(part 1 of 3)
# Autodesk Inventor assembly: Почти готово_CPY
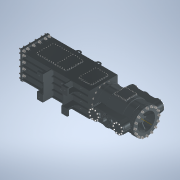
[picture p0: Inventor's stored thumbnail of the model, 180x180]
Saved by Autodesk Inventor 2021 (Build 250183000, 183)
## iProperties
Created: 2020-12-08
Part Number: Почти готово_CPY
Document SubType Name: Assembly
Designer: Тимоха
Author: Тимоха
## Documents named in this file (74)
- C:\Users\Тимоха\Desktop\КР Компрессор\compressor\Почти готово_CPY.iam
- C:\Users\Тимоха\Desktop\КР Компрессор\compressor\Фонарь_CPY.ipt
- C:\Users\Тимоха\Desktop\КР Компрессор\compressor\Башмак_CPY.ipt
- C:\Users\Тимоха\Desktop\КР Компрессор\compressor\Втулка палец шатун_CPY.ipt
- C:\Users\Тимоха\Desktop\КР Компрессор\compressor\Втулка под палец_CPY.ipt
- C:\Users\Тимоха\Desktop\КР Компрессор\compressor\Гайка шток_CPY.ipt
- C:\Users\Тимоха\Desktop\КР Компрессор\compressor\Крейцкопф_CPY.ipt
- C:\Users\Тимоха\Desktop\КР Компрессор\compressor\Палец_CPY.ipt
- C:\Users\Тимоха\Desktop\КР Компрессор\compressor\Стопорное кольцо_CPY.ipt
- C:\Users\Тимоха\Desktop\КР Компрессор\compressor\Верхняя часть поршня_CPY.ipt
- C:\Users\Тимоха\Desktop\КР Компрессор\compressor\Втулка_CPY.ipt
- C:\Users\Тимоха\Desktop\КР Компрессор\compressor\Гайка шток-поршень_CPY.ipt
- C:\Users\Тимоха\Desktop\КР Компрессор\compressor\Кольцо поршень-шток верх_CPY.ipt
- C:\Users\Тимоха\Desktop\КР Компрессор\compressor\Кольцо поршень-шток низ_CPY.ipt
- C:\Users\Тимоха\Desktop\КР Компрессор\compressor\Кольцо поршня_CPY.ipt
- C:\Users\Тимоха\Desktop\КР Компрессор\compressor\Кольцо сальника_CPY.ipt
- C:\Users\Тимоха\Desktop\КР Компрессор\compressor\Корпус дросселя_CPY.ipt
- C:\Users\Тимоха\Desktop\КР Компрессор\compressor\Корпус сальника_CPY.ipt
- C:\Users\Тимоха\Desktop\КР Компрессор\compressor\Крышка стакана_CPY.ipt
- C:\Users\Тимоха\Desktop\КР Компрессор\compressor\Крышка цилиндра 1_CPY.ipt
- C:\Users\Тимоха\Desktop\КР Компрессор\compressor\Крышка цилиндра 2_CPY.ipt
- C:\Users\Тимоха\Desktop\КР Компрессор\compressor\Нижняя часть поршня_CPY.ipt
- C:\Users\Тимоха\Desktop\КР Компрессор\compressor\Опорное кольцо_CPY.ipt
- C:\Users\Тимоха\Desktop\КР Компрессор\compressor\Пружина дросселя_CPY.ipt
- C:\Users\Тимоха\Desktop\КР Компрессор\compressor\Пружина сальника_CPY.ipt
- C:\Users\Тимоха\Desktop\КР Компрессор\compressor\Цилиндр2_CPY.ipt
- C:\Users\Тимоха\Desktop\КР Компрессор\compressor\Клапан1_CPY.iam
- C:\Users\Тимоха\Desktop\КР Компрессор\compressor\Прокладка клапана_CPY.ipt
- C:\Users\Тимоха\Desktop\КР Компрессор\compressor\Стакан1_CPY.ipt
- C:\Users\Тимоха\Desktop\КР Компрессор\compressor\Дроссельное кольцо_CPY.ipt
- C:\Users\Тимоха\Desktop\КР Компрессор\compressor\Уплотнительное кольцо_CPY.ipt
- C:\Users\Тимоха\Desktop\КР Компрессор\compressor\Уплотнение фонарь_CPY.ipt
- C:\Users\Тимоха\Desktop\КР Компрессор\compressor\Крышка сальников_CPY.ipt
- C:\Users\Тимоха\Desktop\КР Компрессор\compressor\Корпус маслосъемника_CPY.ipt
- C:\Users\Тимоха\Desktop\КР Компрессор\compressor\Корпус сальника перегородка 1_CPY.ipt
- C:\Users\Тимоха\Desktop\КР Компрессор\compressor\Крышка перегородки11_CPY.ipt
- C:\Users\Тимоха\Desktop\КР Компрессор\compressor\Крышка перегородки12_CPY.ipt
- C:\Users\Тимоха\Desktop\КР Компрессор\compressor\Крышка перегородки21_CPY.ipt
- C:\Users\Тимоха\Desktop\КР Компрессор\compressor\Крышка перегородки22_CPY.ipt
- C:\Users\Тимоха\Desktop\КР Компрессор\compressor\Маслосъемная пружина_CPY.ipt
- C:\Users\Тимоха\Desktop\КР Компрессор\compressor\Маслосъемное кольцо_CPY.ipt
- C:\Users\Тимоха\Desktop\КР Компрессор\compressor\Придав перегородки1_CPY.ipt
- C:\Users\Тимоха\Desktop\КР Компрессор\compressor\Фланецгайка_CPY.ipt
- C:\Users\Тимоха\Desktop\КР Компрессор\compressor\Шток_CPY.ipt
- C:\Users\Тимоха\Desktop\КР Компрессор\compressor\Прокладка крейцкопф_CPY.ipt
- C:\Users\Тимоха\Documents\Inventor\Content Center Files\R2021\ru-RU\Stud GOST 22038-76\Шпилька M24-6g×70 ГОСТ 22038-76.ipt
- C:\Users\Тимоха\Documents\Inventor\Content Center Files\R2021\ru-RU\Nut GOST 15524-70\Гайка M24-6H ГОСТ 15524-70.ipt
- C:\Users\Тимоха\Documents\Inventor\Content Center Files\R2021\ru-RU\GOST 11371-78  A\Шайба 24 ГОСТ 11371-78.ipt
- C:\Users\Тимоха\Documents\Inventor\Content Center Files\R2021\ru-RU\GOST 15521-70\Гайка M20-6H ГОСТ 15521-70.ipt
- C:\Users\Тимоха\Documents\Inventor\Content Center Files\R2021\ru-RU\Stud GOST 22034-76\Шпилька M20-6g×50 ГОСТ 22034-76.ipt
- C:\Users\Тимоха\Documents\Inventor\Content Center Files\R2021\ru-RU\GOST 10450-78\Шайба 19 ГОСТ 10450-78.ipt
- C:\Users\Тимоха\Documents\Inventor\Content Center Files\R2021\ru-RU\Stud GOST 22038-76\Шпилька M20-6g×85 ГОСТ 22038-76.ipt
- C:\Users\Тимоха\Documents\Inventor\Content Center Files\R2021\ru-RU\GOST 10450-78\Шайба 21 ГОСТ 10450-78.ipt
- C:\Users\Тимоха\Documents\Inventor\Content Center Files\R2021\ru-RU\Nut GOST 15524-70\Гайка M20-6H ГОСТ 15524-70.ipt
- C:\Users\Тимоха\Documents\Inventor\Content Center Files\R2021\ru-RU\GOST 11738-84\Винт M10-6gx35 ГОСТ 11738-84.ipt
- C:\Users\Тимоха\Documents\Inventor\Content Center Files\R2021\ru-RU\GOST 11371-78  A\Шайба 12 ГОСТ 11371-78.ipt
- C:\Users\Тимоха\Documents\Inventor\Content Center Files\R2021\ru-RU\GOST 11738-84\Винт M10-6gx30 ГОСТ 11738-84.ipt
- C:\Users\Тимоха\Documents\Inventor\Content Center Files\R2021\ru-RU\GOST 11738-84\Винт M10-6gx25 ГОСТ 11738-84.ipt
- C:\Users\Тимоха\Documents\Inventor\Content Center Files\R2021\ru-RU\Stud GOST 22038-76\Шпилька M24-6g×80 ГОСТ 22038-76.ipt
- C:\Users\Тимоха\Documents\Inventor\Content Center Files\R2021\ru-RU\GOST 11371-78  A\Шайба 27 ГОСТ 11371-78.ipt
- C:\Users\Тимоха\Desktop\КР Компрессор\compressor\Крышка стакана_MIR_CPY.ipt
- C:\Users\Тимоха\Desktop\КР Компрессор\compressor\Деталь5_CPY.ipt
- C:\Users\Тимоха\Desktop\КР Компрессор\compressor\Деталь6_CPY.ipt
- C:\Users\Тимоха\Documents\Inventor\Content Center Files\R2021\ru-RU\GOST 11371-78  A\Шайба 22 ГОСТ 11371-78.ipt
- C:\Users\Тимоха\Documents\Inventor\Content Center Files\R2021\ru-RU\Bolt GOST R 50274-92\Болт M8-6g×16-F ГОСТ Р 50274-92.ipt
- C:\Users\Тимоха\Desktop\КР Компрессор\compressor\Крышка фонаря 1_CPY.ipt
- C:\Users\Тимоха\Desktop\КР Компрессор\compressor\Крышка фонаря 2_CPY.ipt
- C:\Users\Тимоха\Desktop\КР Компрессор\compressor\Прокладка крышки фонаря 1_CPY.ipt
- C:\Users\Тимоха\Desktop\КР Компрессор\compressor\Прокладка крышки фонаря 2_CPY.ipt
- C:\Users\Тимоха\Desktop\КР Компрессор\compressor\Крышка фонаря 1_MIR_CPY.ipt
- C:\Users\Тимоха\Desktop\КР Компрессор\compressor\Крышка фонаря 2_MIR_CPY.ipt
- C:\Users\Тимоха\Desktop\КР Компрессор\compressor\Прокладка крышки фонаря 1_MIR_CPY.ipt
- C:\Users\Тимоха\Desktop\КР Компрессор\compressor\Прокладка крышки фонаря 2_MIR_CPY.ipt
- C:\Users\Тимоха\Desktop\КР Компрессор\compressor\Маслоотражательное кольцо_CPY.ipt
## Components (741 placed, 73 different names)
1. Фонарь_CPY:1 — Заподлицо:5, Заподлицо:4, Заподлицо:7, Заподлицо:6, Цилиндрический:2, Жесткий:70, Жесткий:69, Жесткий:94, Жесткий:98, Жесткий:97, Жесткий:106, Жесткий:127, Жесткий:163, Жесткий:165, Жесткий:166, Жесткий:164, Жесткий:171, Жесткий:173, Жесткий:174, Жесткий:172, Жесткий:169, Жесткий:167, Жесткий:170, Жесткий:168, Жесткий:192, Жесткий:197, Жесткий:191, Жесткий:196, Жесткий:194, Жесткий:193, Жесткий:195
2. Башмак_CPY:1 — Цилиндрический:2, Жесткий:4
3. Втулка палец шатун_CPY:1 — Жесткий:3
4. Втулка под палец_CPY:1 — Жесткий:1, С поворотом:1
5. Гайка шток_CPY:1 — Жесткий:110
6. Крейцкопф_CPY:1 — Жесткий:4, Жесткий:1, Жесткий:2, Жесткий:5, Жесткий:206, Жесткий:208, Жесткий:209
7. Втулка под палец_CPY:2 — Жесткий:3, Жесткий:2
8. Башмак_CPY:2 — Жесткий:5
9. Палец_CPY:1 — С поворотом:1, Жесткий:7, Жесткий:6
10. Стопорное кольцо_CPY:1 — Жесткий:7
11. Стопорное кольцо_CPY:2 — Жесткий:6
12. Верхняя часть поршня_CPY:1 — Совмещение:1, Жесткий:13, Жесткий:9, Жесткий:8, Жесткий:20
13. Втулка_CPY:1 — Жесткий:16, Жесткий:15, Цилиндрический:1
14. Гайка шток-поршень_CPY:1 — Жесткий:14, Жесткий:107
15. Кольцо поршень-шток верх_CPY:1 — Жесткий:14, Жесткий:13
16. Кольцо поршень-шток низ_CPY:1 — Жесткий:12
17. Кольцо поршня_CPY:1 — Жесткий:9
18. Кольцо сальника_CPY:1 — Жесткий:27, Жесткий:31, Жесткий:30
19. Корпус дросселя_CPY:1 — С поворотом:3, Жесткий:26, Жесткий:62
20. Корпус сальника_CPY:1 — С поворотом:3, Жесткий:32, Жесткий:57
21. Крышка стакана_CPY:1 — Жесткий:23
22. Крышка цилиндра 1_CPY:1 — Совмещение:1, Жесткий:16, Жесткий:112
23. Крышка цилиндра 2_CPY:1 — Жесткий:70, Жесткий:79, Жесткий:61, Жесткий:78, Жесткий:125
24. Нижняя часть поршня_CPY:1 — Жесткий:12, Жесткий:8, Жесткий:21, Жесткий:11, Жесткий:10
25. Опорное кольцо_CPY:1 — Жесткий:21
26. Пружина дросселя_CPY:1 — Жесткий:25
27. Пружина сальника_CPY:1 — Жесткий:27
28. Цилиндр2_CPY:1 — Заподлицо:2, Жесткий:79, Жесткий:23, Жесткий:15, Жесткий:80, Жесткий:18, Жесткий:81, Жесткий:111, Жесткий:116, Жесткий:115, Жесткий:117, Жесткий:118, Жесткий:119, Жесткий:122, Жесткий:202, Жесткий:204
29. Кольцо поршня_CPY:2 — Жесткий:11
30. Кольцо поршня_CPY:3 — Цилиндрический:1, Жесткий:10
31. Клапан1_CPY:1 [sub-assembly] — Жесткий:80
32. Прокладка клапана_CPY:1 — Жесткий:18
33. Стакан1_CPY:1 — Жесткий:81
34. Опорное кольцо_CPY:2 — Жесткий:20
35. Дроссельное кольцо_CPY:1 — Жесткий:26, Жесткий:25
36. Кольцо сальника_CPY:2 — Жесткий:32, Жесткий:31, Жесткий:28
37. Пружина сальника_CPY:2 — Жесткий:28
38. Кольцо сальника_CPY:3 — Жесткий:30, Жесткий:29
39. Пружина сальника_CPY:3 — Жесткий:29
40. Кольцо сальника_CPY:4 — Жесткий:33, Жесткий:37, Жесткий:36
41. Корпус сальника_CPY:2 — Жесткий:57, Жесткий:38, Жесткий:58
42. Пружина сальника_CPY:4 — Жесткий:33
43. Кольцо сальника_CPY:5 — Жесткий:38, Жесткий:37, Жесткий:34
44. Пружина сальника_CPY:5 — Жесткий:34
45. Кольцо сальника_CPY:6 — Жесткий:36, Жесткий:35
46. Пружина сальника_CPY:6 — Жесткий:35
47. Кольцо сальника_CPY:7 — Жесткий:39, Жесткий:43, Жесткий:42
48. Корпус сальника_CPY:3 — Жесткий:58, Жесткий:44, Жесткий:59
49. Пружина сальника_CPY:7 — Жесткий:39
50. Кольцо сальника_CPY:8 — Жесткий:44, Жесткий:43, Жесткий:40
51. Пружина сальника_CPY:8 — Жесткий:40
52. Кольцо сальника_CPY:9 — Жесткий:42, Жесткий:41
53. Пружина сальника_CPY:9 — Жесткий:41
54. Кольцо сальника_CPY:10 — Жесткий:45, Жесткий:49, Жесткий:48
55. Корпус сальника_CPY:4 — Жесткий:59, Жесткий:50, Жесткий:60
56. Пружина сальника_CPY:10 — Жесткий:45
57. Кольцо сальника_CPY:11 — Жесткий:50, Жесткий:49, Жесткий:46
58. Пружина сальника_CPY:11 — Жесткий:46
59. Кольцо сальника_CPY:12 — Жесткий:48, Жесткий:47
60. Пружина сальника_CPY:12 — Жесткий:47
61. Кольцо сальника_CPY:13 — Жесткий:51, Жесткий:55, Жесткий:54
62. Корпус сальника_CPY:5 — Жесткий:60, Жесткий:56, Жесткий:77
63. Пружина сальника_CPY:13 — Жесткий:51
64. Кольцо сальника_CPY:14 — Жесткий:56, Жесткий:55, Жесткий:52
65. Пружина сальника_CPY:14 — Жесткий:52
66. Кольцо сальника_CPY:15 — Жесткий:54, Жесткий:53
67. Пружина сальника_CPY:15 — Жесткий:53
68. Уплотнительное кольцо_CPY:1 — Жесткий:62, Жесткий:61
69. Кольцо сальника_CPY:16 — Жесткий:63, Жесткий:67, Жесткий:66
70. Пружина сальника_CPY:16 — Жесткий:63
71. Кольцо сальника_CPY:17 — Жесткий:67, Жесткий:64, Жесткий:103
72. Пружина сальника_CPY:17 — Жесткий:64
73. Кольцо сальника_CPY:18 — Жесткий:66, Жесткий:65
74. Пружина сальника_CPY:18 — Жесткий:65
75. Уплотнение фонарь_CPY:1 — Жесткий:69
76. Кольцо сальника_CPY:19 — Жесткий:71, Жесткий:75, Жесткий:74
77. Корпус сальника_CPY:6 — Жесткий:77, Жесткий:76
78. Пружина сальника_CPY:19 — Жесткий:71
79. Кольцо сальника_CPY:20 — Жесткий:76, Жесткий:75, Жесткий:72
80. Пружина сальника_CPY:20 — Жесткий:72
81. Кольцо сальника_CPY:21 — Жесткий:74, Жесткий:73
82. Пружина сальника_CPY:21 — Жесткий:73
83. Крышка сальников_CPY:1 — Жесткий:78
84. Корпус маслосъемника_CPY:1 — Жесткий:104, Жесткий:102
85. Корпус сальника перегородка 1_CPY:1 — Жесткий:95, Жесткий:96, Жесткий:87, Жесткий:93
86. Крышка перегородки11_CPY:1 — Жесткий:95, Жесткий:94
87. Крышка перегородки12_CPY:1 — Жесткий:96, Жесткий:128
88. Крышка перегородки21_CPY:1 — Жесткий:104, Жесткий:103, Жесткий:98, Жесткий:105
89. Крышка перегородки22_CPY:1 — Жесткий:105, Жесткий:130
90. Маслосъемная пружина_CPY:1 — Жесткий:99
91. Маслосъемное кольцо_CPY:1 — Жесткий:99, Жесткий:101
92. Придав перегородки1_CPY:1 — Жесткий:97, Жесткий:134
93. Кольцо сальника_CPY:22 — Жесткий:82, Жесткий:86, Жесткий:85
94. Пружина сальника_CPY:22 — Жесткий:82
95. Кольцо сальника_CPY:23 — Жесткий:87, Жесткий:86, Жесткий:83
96. Пружина сальника_CPY:23 — Жесткий:83
97. Кольцо сальника_CPY:24 — Жесткий:85, Жесткий:84
98. Пружина сальника_CPY:24 — Жесткий:84
99. Кольцо сальника_CPY:25 — Жесткий:88, Жесткий:92, Жесткий:91
100. Пружина сальника_CPY:25 — Жесткий:88
101. Кольцо сальника_CPY:26 — Жесткий:93, Жесткий:92, Жесткий:89
102. Пружина сальника_CPY:26 — Жесткий:89
103. Кольцо сальника_CPY:27 — Жесткий:91, Жесткий:90
104. Пружина сальника_CPY:27 — Жесткий:90
105. Маслосъемная пружина_CPY:2 — Жесткий:100
106. Маслосъемное кольцо_CPY:2 — Жесткий:102, Жесткий:101, Жесткий:100
107. Придав перегородки1_CPY:2 — Жесткий:106, Жесткий:132
108. Фланецгайка_CPY:1 — Жесткий:207
109. Шток_CPY:1 — Жесткий:110, Жесткий:107, Жесткий:404
110. Прокладка крейцкопф_CPY:1 — Жесткий:207, Жесткий:206
111. Шпилька ГОСТ 22038-76 M24-6g×70:2 — Жесткий:114
112. Гайка ГОСТ 15524-70 M24:2 — Жесткий:114
113. Шайба  ГОСТ 11371-78 25:2 — Совмещение:2
114. Шпилька ГОСТ 22038-76 M24-6g×70:3
115. Гайка ГОСТ 15524-70 M24:3
116. Шайба  ГОСТ 11371-78 25:3
117. Шпилька ГОСТ 22038-76 M24-6g×70:4
118. Гайка ГОСТ 15524-70 M24:4
119. Шайба  ГОСТ 11371-78 25:4
120. Шпилька ГОСТ 22038-76 M24-6g×70:5
121. Гайка ГОСТ 15524-70 M24:5
122. Шайба  ГОСТ 11371-78 25:5
123. Шпилька ГОСТ 22038-76 M24-6g×70:6
124. Гайка ГОСТ 15524-70 M24:6
125. Шайба  ГОСТ 11371-78 25:6
126. Шпилька ГОСТ 22038-76 M24-6g×70:7
127. Гайка ГОСТ 15524-70 M24:7
128. Шайба  ГОСТ 11371-78 25:7
129. Шпилька ГОСТ 22038-76 M24-6g×70:8
130. Гайка ГОСТ 15524-70 M24:8
131. Шайба  ГОСТ 11371-78 25:8
132. Шпилька ГОСТ 22038-76 M24-6g×70:9
133. Гайка ГОСТ 15524-70 M24:9
134. Шайба  ГОСТ 11371-78 25:9
135. Шпилька ГОСТ 22038-76 M24-6g×70:10
136. Гайка ГОСТ 15524-70 M24:10
137. Шайба  ГОСТ 11371-78 25:10
138. Шпилька ГОСТ 22038-76 M24-6g×70:11
139. Гайка ГОСТ 15524-70 M24:11
140. Шайба  ГОСТ 11371-78 25:11
141. Шпилька ГОСТ 22038-76 M24-6g×70:12
142. Гайка ГОСТ 15524-70 M24:12
143. Шайба  ГОСТ 11371-78 25:12
144. Шпилька ГОСТ 22038-76 M24-6g×70:13
145. Гайка ГОСТ 15524-70 M24:13
146. Шайба  ГОСТ 11371-78 25:13
147. Шпилька ГОСТ 22038-76 M24-6g×70:14
148. Гайка ГОСТ 15524-70 M24:14
149. Шайба  ГОСТ 11371-78 25:14
150. Шпилька ГОСТ 22038-76 M24-6g×70:15
151. Гайка ГОСТ 15524-70 M24:15
152. Шайба  ГОСТ 11371-78 25:15
153. Шпилька ГОСТ 22038-76 M24-6g×70:16
154. Гайка ГОСТ 15524-70 M24:16
155. Шайба  ГОСТ 11371-78 25:16
156. Шпилька ГОСТ 22038-76 M24-6g×70:17
157. Гайка ГОСТ 15524-70 M24:17
158. Шайба  ГОСТ 11371-78 25:17
159. Клапан1_CPY:2 [sub-assembly] — Жесткий:116
160. Прокладка клапана_CPY:2 — Жесткий:115
161. Стакан1_CPY:2 — Жесткий:117
162. Крышка стакана_CPY:2 — Жесткий:118
163. Шпилька ГОСТ 22038-76 M24-6g×80:1 — Жесткий:138, Жесткий:137
164. Гайка ГОСТ 15524-70 M24:18 — Жесткий:138
165. Шайба  ГОСТ 11371-78 28:1 — Жесткий:137
166. Шпилька ГОСТ 22038-76 M24-6g×80:2 — Жесткий:140, Жесткий:139
167. Гайка ГОСТ 15524-70 M24:19 — Жесткий:140
168. Шайба  ГОСТ 11371-78 28:2 — Жесткий:163, Жесткий:139
169. Шпилька ГОСТ 22038-76 M24-6g×80:3 — Жесткий:142, Жесткий:141
170. Гайка ГОСТ 15524-70 M24:20 — Жесткий:142
171. Шайба  ГОСТ 11371-78 28:3 — Жесткий:165, Жесткий:141
172. Шпилька ГОСТ 22038-76 M24-6g×80:4 — Жесткий:144, Жесткий:143
173. Гайка ГОСТ 15524-70 M24:21 — Жесткий:144
174. Шайба  ГОСТ 11371-78 28:4 — Жесткий:166, Жесткий:143
175. Шпилька ГОСТ 22038-76 M24-6g×80:5 — Жесткий:146, Жесткий:145
176. Гайка ГОСТ 15524-70 M24:22 — Жесткий:146
177. Шайба  ГОСТ 11371-78 28:5 — Жесткий:164, Жесткий:145
178. Шпилька ГОСТ 22038-76 M24-6g×80:6 — Жесткий:148, Жесткий:147
179. Гайка ГОСТ 15524-70 M24:23 — Жесткий:148
180. Шайба  ГОСТ 11371-78 28:6 — Жесткий:171, Жесткий:147
181. Шпилька ГОСТ 22038-76 M24-6g×80:7 — Жесткий:150, Жесткий:149
182. Гайка ГОСТ 15524-70 M24:24 — Жесткий:150
183. Шайба  ГОСТ 11371-78 28:7 — Жесткий:173, Жесткий:149
184. Шпилька ГОСТ 22038-76 M24-6g×80:8 — Жесткий:152, Жесткий:151
185. Гайка ГОСТ 15524-70 M24:25 — Жесткий:152
186. Шайба  ГОСТ 11371-78 28:8 — Жесткий:174, Жесткий:151
187. Шпилька ГОСТ 22038-76 M24-6g×80:9 — Жесткий:154, Жесткий:153
188. Гайка ГОСТ 15524-70 M24:26 — Жесткий:154
189. Шайба  ГОСТ 11371-78 28:9 — Жесткий:172, Жесткий:153
190. Шпилька ГОСТ 22038-76 M24-6g×80:10 — Жесткий:156, Жесткий:155
191. Гайка ГОСТ 15524-70 M24:27 — Жесткий:156
192. Шайба  ГОСТ 11371-78 28:10 — Жесткий:169, Жесткий:155
193. Шпилька ГОСТ 22038-76 M24-6g×80:11 — Жесткий:158, Жесткий:157
194. Гайка ГОСТ 15524-70 M24:28 — Жесткий:158
195. Шайба  ГОСТ 11371-78 28:11 — Жесткий:167, Жесткий:157
196. Шпилька ГОСТ 22038-76 M24-6g×80:12 — Жесткий:160, Жесткий:159
197. Гайка ГОСТ 15524-70 M24:29 — Жесткий:160
198. Шайба  ГОСТ 11371-78 28:12 — Жесткий:170, Жесткий:159
199. Шпилька ГОСТ 22038-76 M24-6g×80:13 — Жесткий:162, Жесткий:161
200. Гайка ГОСТ 15524-70 M24:30 — Жесткий:162
201. Шайба  ГОСТ 11371-78 28:13 — Жесткий:168, Жесткий:161
202. Шпилька ГОСТ 22038-76 M24-6g×80:14 — Жесткий:176, Жесткий:175
203. Гайка ГОСТ 15524-70 M24:31 — Жесткий:176
204. Шайба  ГОСТ 11371-78 28:14 — Жесткий:192, Жесткий:175
205. Шпилька ГОСТ 22038-76 M24-6g×80:15 — Жесткий:178, Жесткий:177
206. Гайка ГОСТ 15524-70 M24:32 — Жесткий:178
207. Шайба  ГОСТ 11371-78 28:15 — Жесткий:197, Жесткий:177
208. Шпилька ГОСТ 22038-76 M24-6g×80:16 — Жесткий:180, Жесткий:179
209. Гайка ГОСТ 15524-70 M24:33 — Жесткий:180
210. Шайба  ГОСТ 11371-78 28:16 — Жесткий:191, Жесткий:179
211. Шпилька ГОСТ 22038-76 M24-6g×80:17 — Жесткий:184, Жесткий:183
212. Гайка ГОСТ 15524-70 M24:34 — Жесткий:184
213. Шайба  ГОСТ 11371-78 28:17 — Жесткий:196, Жесткий:183
214. Шпилька ГОСТ 22038-76 M24-6g×80:18 — Жесткий:186, Жесткий:185
215. Гайка ГОСТ 15524-70 M24:35 — Жесткий:186
216. Шайба  ГОСТ 11371-78 28:18 — Жесткий:194, Жесткий:185
217. Шпилька ГОСТ 22038-76 M24-6g×80:19 — Жесткий:188, Жесткий:187
218. Гайка ГОСТ 15524-70 M24:36 — Жесткий:188
219. Шайба  ГОСТ 11371-78 28:19 — Жесткий:193, Жесткий:187
220. Шпилька ГОСТ 22038-76 M24-6g×80:20 — Жесткий:190, Жесткий:189
221. Гайка ГОСТ 15524-70 M24:37 — Жесткий:190
222. Шайба  ГОСТ 11371-78 28:20 — Жесткий:195, Жесткий:189
223. Крышка стакана_MIR_CPY:1
224. Крышка стакана_MIR_CPY:2
225. Деталь5_CPY:1 — Жесткий:202, Жесткий:203
226. Деталь6_CPY:1 — Заподлицо:3, Жесткий:203, Жесткий:239, Жесткий:233, Жесткий:232, Жесткий:214, Жесткий:215, Жесткий:223, Жесткий:222, Жесткий:240, Жесткий:238, Жесткий:236, Жесткий:218, Жесткий:217, Жесткий:216, Жесткий:237, Жесткий:235, Жесткий:234, Жесткий:227, Жесткий:226, Жесткий:225, Жесткий:241, Жесткий:244, Жесткий:231, Жесткий:229, Жесткий:228, Жесткий:224, Жесткий:243, Жесткий:242, Жесткий:219, Жесткий:221, Жесткий:220, Жесткий:245, Жесткий:230
227. Деталь5_CPY:2 — Жесткий:204, Жесткий:205
228. Деталь6_CPY:2 — Жесткий:205
229. Шпилька ГОСТ 22038-76 M20-6g×85:2 — Жесткий:208, Жесткий:211, Жесткий:210
230. Шпилька ГОСТ 22038-76 M20-6g×85:3 — Жесткий:209, Жесткий:213, Жесткий:212
231. Гайка ГОСТ 15524-70 M20:2 — Жесткий:211
232. Шайба  ГОСТ 11371-78 23:1 — Жесткий:210
233. Гайка ГОСТ 15524-70 M20:3 — Жесткий:213
234. Шайба  ГОСТ 11371-78 23:2 — Жесткий:212
235. Болт ГОСТ Р 50274-92 M8-6g×16-F:1 — Жесткий:239
236. Болт ГОСТ Р 50274-92 M8-6g×16-F:2 — Жесткий:233
237. Болт ГОСТ Р 50274-92 M8-6g×16-F:3 — Жесткий:232
238. Болт ГОСТ Р 50274-92 M8-6g×16-F:4 — Жесткий:214
239. Болт ГОСТ Р 50274-92 M8-6g×16-F:5 — Жесткий:215
240. Болт ГОСТ Р 50274-92 M8-6g×16-F:6 — Жесткий:223
241. Болт ГОСТ Р 50274-92 M8-6g×16-F:7 — Жесткий:222
242. Болт ГОСТ Р 50274-92 M8-6g×16-F:8 — Жесткий:240
243. Болт ГОСТ Р 50274-92 M8-6g×16-F:9 — Жесткий:238
244. Болт ГОСТ Р 50274-92 M8-6g×16-F:10 — Жесткий:236
245. Болт ГОСТ Р 50274-92 M8-6g×16-F:11 — Жесткий:218
246. Болт ГОСТ Р 50274-92 M8-6g×16-F:12 — Жесткий:217
247. Болт ГОСТ Р 50274-92 M8-6g×16-F:13 — Жесткий:216
248. Болт ГОСТ Р 50274-92 M8-6g×16-F:14 — Жесткий:237
249. Болт ГОСТ Р 50274-92 M8-6g×16-F:15 — Жесткий:235
250. Болт ГОСТ Р 50274-92 M8-6g×16-F:16 — Жесткий:234
251. Болт ГОСТ Р 50274-92 M8-6g×16-F:17 — Жесткий:227
252. Болт ГОСТ Р 50274-92 M8-6g×16-F:18 — Жесткий:226
253. Болт ГОСТ Р 50274-92 M8-6g×16-F:19 — Жесткий:225
254. Болт ГОСТ Р 50274-92 M8-6g×16-F:20 — Жесткий:241
255. Болт ГОСТ Р 50274-92 M8-6g×16-F:21 — Жесткий:244
256. Болт ГОСТ Р 50274-92 M8-6g×16-F:22 — Жесткий:231
257. Болт ГОСТ Р 50274-92 M8-6g×16-F:23 — Жесткий:229
258. Болт ГОСТ Р 50274-92 M8-6g×16-F:24 — Жесткий:228
259. Болт ГОСТ Р 50274-92 M8-6g×16-F:25 — Жесткий:224
260. Болт ГОСТ Р 50274-92 M8-6g×16-F:26 — Жесткий:243
261. Болт ГОСТ Р 50274-92 M8-6g×16-F:27 — Жесткий:242
262. Болт ГОСТ Р 50274-92 M8-6g×16-F:28 — Жесткий:219
263. Болт ГОСТ Р 50274-92 M8-6g×16-F:29 — Жесткий:221
264. Болт ГОСТ Р 50274-92 M8-6g×16-F:30 — Жесткий:220
265. Болт ГОСТ Р 50274-92 M8-6g×16-F:31 — Жесткий:245
266. Болт ГОСТ Р 50274-92 M8-6g×16-F:32 — Жесткий:230
267. Болт ГОСТ Р 50274-92 M8-6g×16-F:33
268. Болт ГОСТ Р 50274-92 M8-6g×16-F:34
269. Болт ГОСТ Р 50274-92 M8-6g×16-F:35
270. Болт ГОСТ Р 50274-92 M8-6g×16-F:36
271. Болт ГОСТ Р 50274-92 M8-6g×16-F:37
272. Болт ГОСТ Р 50274-92 M8-6g×16-F:38
273. Болт ГОСТ Р 50274-92 M8-6g×16-F:39
274. Болт ГОСТ Р 50274-92 M8-6g×16-F:40
275. Болт ГОСТ Р 50274-92 M8-6g×16-F:41
276. Болт ГОСТ Р 50274-92 M8-6g×16-F:42
277. Болт ГОСТ Р 50274-92 M8-6g×16-F:43
278. Болт ГОСТ Р 50274-92 M8-6g×16-F:44
279. Болт ГОСТ Р 50274-92 M8-6g×16-F:45
280. Болт ГОСТ Р 50274-92 M8-6g×16-F:46
281. Болт ГОСТ Р 50274-92 M8-6g×16-F:47
282. Болт ГОСТ Р 50274-92 M8-6g×16-F:48
283. Болт ГОСТ Р 50274-92 M8-6g×16-F:49
284. Болт ГОСТ Р 50274-92 M8-6g×16-F:50
285. Болт ГОСТ Р 50274-92 M8-6g×16-F:51
286. Болт ГОСТ Р 50274-92 M8-6g×16-F:52
287. Болт ГОСТ Р 50274-92 M8-6g×16-F:53
288. Болт ГОСТ Р 50274-92 M8-6g×16-F:54
289. Болт ГОСТ Р 50274-92 M8-6g×16-F:55
290. Болт ГОСТ Р 50274-92 M8-6g×16-F:56
291. Болт ГОСТ Р 50274-92 M8-6g×16-F:57
292. Болт ГОСТ Р 50274-92 M8-6g×16-F:58
293. Болт ГОСТ Р 50274-92 M8-6g×16-F:59
294. Болт ГОСТ Р 50274-92 M8-6g×16-F:60
295. Болт ГОСТ Р 50274-92 M8-6g×16-F:61
296. Болт ГОСТ Р 50274-92 M8-6g×16-F:62
297. Болт ГОСТ Р 50274-92 M8-6g×16-F:63
298. Болт ГОСТ Р 50274-92 M8-6g×16-F:64
299. Крышка фонаря 1_CPY:1 — Жесткий:246, Жесткий:249, Жесткий:248, Жесткий:250, Жесткий:251, Жесткий:254, Жесткий:252, Жесткий:258, Жесткий:256, Жесткий:255, Жесткий:253, Жесткий:267, Жесткий:266, Жесткий:269, Жесткий:265, Жесткий:273, Жесткий:271, Жесткий:270, Жесткий:268, Жесткий:257, Жесткий:259, Жесткий:261, Жесткий:264, Жесткий:263, Жесткий:262, Жесткий:260, Жесткий:274, Жесткий:272, Жесткий:275
300. Крышка фонаря 2_CPY:1 — Жесткий:247, Жесткий:280, Жесткий:281, Жесткий:279, Жесткий:276, Жесткий:295, Жесткий:296, Жесткий:282, Жесткий:278, Жесткий:277, Жесткий:308, Жесткий:317, Жесткий:318, Жесткий:316, Жесткий:310, Жесткий:294, Жесткий:311, Жесткий:307, Жесткий:313, Жесткий:314, Жесткий:315, Жесткий:293, Жесткий:320, Жесткий:300, Жесткий:299, Жесткий:285, Жесткий:301, Жесткий:291, Жесткий:284, Жесткий:309, Жесткий:289, Жесткий:306, Жесткий:297, Жесткий:312, Жесткий:288, Жесткий:319, Жесткий:303, Жесткий:292, Жесткий:304, Жесткий:305, Жесткий:298, Жесткий:302, Жесткий:283, Жесткий:290, Жесткий:286, Жесткий:287, Жесткий:321, Жесткий:323, Жесткий:322, Жесткий:324
301. Прокладка крышки фонаря 1_CPY:1 — Заподлицо:5, Заподлицо:4, Жесткий:246
302. Прокладка крышки фонаря 2_CPY:1 — Заподлицо:7, Заподлицо:6, Жесткий:247
303. Болт ГОСТ Р 50274-92 M8-6g×16-F:65 — Жесткий:249
304. Болт ГОСТ Р 50274-92 M8-6g×16-F:66 — Жесткий:248
305. Болт ГОСТ Р 50274-92 M8-6g×16-F:67 — Жесткий:250
306. Болт ГОСТ Р 50274-92 M8-6g×16-F:68 — Жесткий:251
307. Болт ГОСТ Р 50274-92 M8-6g×16-F:69 — Жесткий:254
308. Болт ГОСТ Р 50274-92 M8-6g×16-F:70 — Жесткий:252
309. Болт ГОСТ Р 50274-92 M8-6g×16-F:71 — Жесткий:258
310. Болт ГОСТ Р 50274-92 M8-6g×16-F:72 — Жесткий:256
311. Болт ГОСТ Р 50274-92 M8-6g×16-F:73 — Жесткий:255
312. Болт ГОСТ Р 50274-92 M8-6g×16-F:74 — Жесткий:253
313. Болт ГОСТ Р 50274-92 M8-6g×16-F:75 — Жесткий:267
314. Болт ГОСТ Р 50274-92 M8-6g×16-F:76 — Жесткий:266
315. Болт ГОСТ Р 50274-92 M8-6g×16-F:77 — Жесткий:269
316. Болт ГОСТ Р 50274-92 M8-6g×16-F:78 — Жесткий:265
317. Болт ГОСТ Р 50274-92 M8-6g×16-F:79 — Жесткий:273
318. Болт ГОСТ Р 50274-92 M8-6g×16-F:80 — Жесткий:271
319. Болт ГОСТ Р 50274-92 M8-6g×16-F:81 — Жесткий:270
320. Болт ГОСТ Р 50274-92 M8-6g×16-F:82 — Жесткий:268
321. Болт ГОСТ Р 50274-92 M8-6g×16-F:83 — Жесткий:257
322. Болт ГОСТ Р 50274-92 M8-6g×16-F:84 — Жесткий:259
323. Болт ГОСТ Р 50274-92 M8-6g×16-F:85 — Жесткий:261
324. Болт ГОСТ Р 50274-92 M8-6g×16-F:86 — Жесткий:264
325. Болт ГОСТ Р 50274-92 M8-6g×16-F:87 — Жесткий:263
326. Болт ГОСТ Р 50274-92 M8-6g×16-F:88 — Жесткий:262
327. Болт ГОСТ Р 50274-92 M8-6g×16-F:89 — Жесткий:260
328. Болт ГОСТ Р 50274-92 M8-6g×16-F:90 — Жесткий:280
329. Болт ГОСТ Р 50274-92 M8-6g×16-F:91 — Жесткий:281
330. Болт ГОСТ Р 50274-92 M8-6g×16-F:92 — Жесткий:279
331. Болт ГОСТ Р 50274-92 M8-6g×16-F:93 — Жесткий:276
332. Болт ГОСТ Р 50274-92 M8-6g×16-F:94 — Жесткий:295
333. Болт ГОСТ Р 50274-92 M8-6g×16-F:95 — Жесткий:296
334. Болт ГОСТ Р 50274-92 M8-6g×16-F:96 — Жесткий:282
335. Болт ГОСТ Р 50274-92 M8-6g×16-F:97 — Жесткий:278
336. Болт ГОСТ Р 50274-92 M8-6g×16-F:98 — Жесткий:277
337. Болт ГОСТ Р 50274-92 M8-6g×16-F:99 — Жесткий:308
338. Болт ГОСТ Р 50274-92 M8-6g×16-F:100 — Жесткий:274
339. Болт ГОСТ Р 50274-92 M8-6g×16-F:101 — Жесткий:272
340. Болт ГОСТ Р 50274-92 M8-6g×16-F:102 — Жесткий:317
341. Болт ГОСТ Р 50274-92 M8-6g×16-F:103 — Жесткий:318
342. Болт ГОСТ Р 50274-92 M8-6g×16-F:104 — Жесткий:316
343. Болт ГОСТ Р 50274-92 M8-6g×16-F:105 — Жесткий:275
344. Болт ГОСТ Р 50274-92 M8-6g×16-F:106 — Жесткий:310
345. Болт ГОСТ Р 50274-92 M8-6g×16-F:107 — Жесткий:294
346. Болт ГОСТ Р 50274-92 M8-6g×16-F:108 — Жесткий:311
347. Болт ГОСТ Р 50274-92 M8-6g×16-F:109 — Жесткий:307
348. Болт ГОСТ Р 50274-92 M8-6g×16-F:110 — Жесткий:313
349. Болт ГОСТ Р 50274-92 M8-6g×16-F:111 — Жесткий:314
350. Болт ГОСТ Р 50274-92 M8-6g×16-F:112 — Жесткий:315
351. Болт ГОСТ Р 50274-92 M8-6g×16-F:113 — Жесткий:293
352. Болт ГОСТ Р 50274-92 M8-6g×16-F:114 — Жесткий:320
353. Болт ГОСТ Р 50274-92 M8-6g×16-F:115 — Жесткий:300
354. Болт ГОСТ Р 50274-92 M8-6g×16-F:116 — Жесткий:299
355. Болт ГОСТ Р 50274-92 M8-6g×16-F:117 — Жесткий:285
356. Болт ГОСТ Р 50274-92 M8-6g×16-F:118 — Жесткий:301
357. Болт ГОСТ Р 50274-92 M8-6g×16-F:119 — Жесткий:291
358. Болт ГОСТ Р 50274-92 M8-6g×16-F:120 — Жесткий:284
359. Болт ГОСТ Р 50274-92 M8-6g×16-F:121 — Жесткий:309
360. Болт ГОСТ Р 50274-92 M8-6g×16-F:122 — Жесткий:289
361. Болт ГОСТ Р 50274-92 M8-6g×16-F:123 — Жесткий:306
362. Болт ГОСТ Р 50274-92 M8-6g×16-F:124 — Жесткий:297
363. Болт ГОСТ Р 50274-92 M8-6g×16-F:125 — Жесткий:312
364. Болт ГОСТ Р 50274-92 M8-6g×16-F:126 — Жесткий:288
365. Болт ГОСТ Р 50274-92 M8-6g×16-F:127 — Жесткий:319
366. Болт ГОСТ Р 50274-92 M8-6g×16-F:128 — Жесткий:303
367. Болт ГОСТ Р 50274-92 M8-6g×16-F:129 — Жесткий:292
368. Болт ГОСТ Р 50274-92 M8-6g×16-F:130 — Жесткий:304
369. Болт ГОСТ Р 50274-92 M8-6g×16-F:131 — Жесткий:305
370. Болт ГОСТ Р 50274-92 M8-6g×16-F:132 — Жесткий:298
371. Болт ГОСТ Р 50274-92 M8-6g×16-F:133 — Жесткий:302
372. Болт ГОСТ Р 50274-92 M8-6g×16-F:134 — Жесткий:283
373. Болт ГОСТ Р 50274-92 M8-6g×16-F:135 — Жесткий:290
374. Болт ГОСТ Р 50274-92 M8-6g×16-F:136 — Жесткий:286
375. Болт ГОСТ Р 50274-92 M8-6g×16-F:137 — Жесткий:287
376. Болт ГОСТ Р 50274-92 M8-6g×16-F:138 — Жесткий:321
377. Болт ГОСТ Р 50274-92 M8-6g×16-F:139 — Жесткий:323
378. Болт ГОСТ Р 50274-92 M8-6g×16-F:140 — Жесткий:322
379. Болт ГОСТ Р 50274-92 M8-6g×16-F:141 — Жесткий:324
380. Крышка фонаря 1_MIR_CPY:1 — Жесткий:325, Жесткий:327, Жесткий:328, Жесткий:329, Жесткий:330, Жесткий:331, Жесткий:332, Жесткий:333, Жесткий:334, Жесткий:335, Жесткий:336, Жесткий:337, Жесткий:338, Жесткий:339, Жесткий:340, Жесткий:341, Жесткий:342, Жесткий:343, Жесткий:344, Жесткий:345, Жесткий:346, Жесткий:347, Жесткий:348, Жесткий:349, Жесткий:350, Жесткий:351, Жесткий:362, Жесткий:363, Жесткий:367
381. Крышка фонаря 2_MIR_CPY:1 — Жесткий:326, Жесткий:352, Жесткий:353, Жесткий:354, Жесткий:355, Жесткий:356, Жесткий:357, Жесткий:358, Жесткий:359, Жесткий:360, Жесткий:361, Жесткий:364, Жесткий:365, Жесткий:366, Жесткий:368, Жесткий:369, Жесткий:370, Жесткий:371, Жесткий:372, Жесткий:373, Жесткий:374, Жесткий:375, Жесткий:376, Жесткий:377, Жесткий:378, Жесткий:379, Жесткий:380, Жесткий:381, Жесткий:382, Жесткий:383, Жесткий:384, Жесткий:385, Жесткий:386, Жесткий:387, Жесткий:388, Жесткий:389, Жесткий:390, Жесткий:391, Жесткий:392, Жесткий:393, Жесткий:394, Жесткий:395, Жесткий:396, Жесткий:397, Жесткий:398, Жесткий:399, Жесткий:400, Жесткий:401, Жесткий:402, Жесткий:403
382. Прокладка крышки фонаря 1_MIR_CPY:1 — Жесткий:325
383. Прокладка крышки фонаря 2_MIR_CPY:1 — Жесткий:326
384. Болт ГОСТ Р 50274-92 M8-6g×16-F:142 — Жесткий:327
385. Болт ГОСТ Р 50274-92 M8-6g×16-F:143 — Жесткий:328
386. Болт ГОСТ Р 50274-92 M8-6g×16-F:144 — Жесткий:329
387. Болт ГОСТ Р 50274-92 M8-6g×16-F:145 — Жесткий:330
388. Болт ГОСТ Р 50274-92 M8-6g×16-F:146 — Жесткий:331
389. Болт ГОСТ Р 50274-92 M8-6g×16-F:147 — Жесткий:332
390. Болт ГОСТ Р 50274-92 M8-6g×16-F:148 — Жесткий:333
391. Болт ГОСТ Р 50274-92 M8-6g×16-F:149 — Жесткий:334
392. Болт ГОСТ Р 50274-92 M8-6g×16-F:150 — Жесткий:335
393. Болт ГОСТ Р 50274-92 M8-6g×16-F:151 — Жесткий:336
394. Болт ГОСТ Р 50274-92 M8-6g×16-F:152 — Жесткий:337
395. Болт ГОСТ Р 50274-92 M8-6g×16-F:153 — Жесткий:338
396. Болт ГОСТ Р 50274-92 M8-6g×16-F:154 — Жесткий:339
397. Болт ГОСТ Р 50274-92 M8-6g×16-F:155 — Жесткий:340
398. Болт ГОСТ Р 50274-92 M8-6g×16-F:156 — Жесткий:341
399. Болт ГОСТ Р 50274-92 M8-6g×16-F:157 — Жесткий:342
400. Болт ГОСТ Р 50274-92 M8-6g×16-F:158 — Жесткий:343
401. Болт ГОСТ Р 50274-92 M8-6g×16-F:159 — Жесткий:344
402. Болт ГОСТ Р 50274-92 M8-6g×16-F:160 — Жесткий:345
403. Болт ГОСТ Р 50274-92 M8-6g×16-F:161 — Жесткий:346
404. Болт ГОСТ Р 50274-92 M8-6g×16-F:162 — Жесткий:347
405. Болт ГОСТ Р 50274-92 M8-6g×16-F:163 — Жесткий:348
406. Болт ГОСТ Р 50274-92 M8-6g×16-F:164 — Жесткий:349
407. Болт ГОСТ Р 50274-92 M8-6g×16-F:165 — Жесткий:350
408. Болт ГОСТ Р 50274-92 M8-6g×16-F:166 — Жесткий:351
409. Болт ГОСТ Р 50274-92 M8-6g×16-F:167 — Жесткий:352
410. Болт ГОСТ Р 50274-92 M8-6g×16-F:168 — Жесткий:353
411. Болт ГОСТ Р 50274-92 M8-6g×16-F:169 — Жесткий:354
412. Болт ГОСТ Р 50274-92 M8-6g×16-F:170 — Жесткий:355
413. Болт ГОСТ Р 50274-92 M8-6g×16-F:171 — Жесткий:356
414. Болт ГОСТ Р 50274-92 M8-6g×16-F:172 — Жесткий:357
415. Болт ГОСТ Р 50274-92 M8-6g×16-F:173 — Жесткий:358
416. Болт ГОСТ Р 50274-92 M8-6g×16-F:174 — Жесткий:359
417. Болт ГОСТ Р 50274-92 M8-6g×16-F:175 — Жесткий:360
418. Болт ГОСТ Р 50274-92 M8-6g×16-F:176 — Жесткий:361
419. Болт ГОСТ Р 50274-92 M8-6g×16-F:177 — Жесткий:362
420. Болт ГОСТ Р 50274-92 M8-6g×16-F:178 — Жесткий:363
421. Болт ГОСТ Р 50274-92 M8-6g×16-F:179 — Жесткий:364
422. Болт ГОСТ Р 50274-92 M8-6g×16-F:180 — Жесткий:365
423. Болт ГОСТ Р 50274-92 M8-6g×16-F:181 — Жесткий:366
424. Болт ГОСТ Р 50274-92 M8-6g×16-F:182 — Жесткий:367
425. Болт ГОСТ Р 50274-92 M8-6g×16-F:183 — Жесткий:368
426. Болт ГОСТ Р 50274-92 M8-6g×16-F:184 — Жесткий:369
427. Болт ГОСТ Р 50274-92 M8-6g×16-F:185 — Жесткий:370
428. Болт ГОСТ Р 50274-92 M8-6g×16-F:186 — Жесткий:371
429. Болт ГОСТ Р 50274-92 M8-6g×16-F:187 — Жесткий:372
430. Болт ГОСТ Р 50274-92 M8-6g×16-F:188 — Жесткий:373
431. Болт ГОСТ Р 50274-92 M8-6g×16-F:189 — Жесткий:374
432. Болт ГОСТ Р 50274-92 M8-6g×16-F:190 — Жесткий:375
433. Болт ГОСТ Р 50274-92 M8-6g×16-F:191 — Жесткий:376
434. Болт ГОСТ Р 50274-92 M8-6g×16-F:192 — Жесткий:377
435. Болт ГОСТ Р 50274-92 M8-6g×16-F:193 — Жесткий:378
436. Болт ГОСТ Р 50274-92 M8-6g×16-F:194 — Жесткий:379
437. Болт ГОСТ Р 50274-92 M8-6g×16-F:195 — Жесткий:380
438. Болт ГОСТ Р 50274-92 M8-6g×16-F:196 — Жесткий:381
439. Болт ГОСТ Р 50274-92 M8-6g×16-F:197 — Жесткий:382
440. Болт ГОСТ Р 50274-92 M8-6g×16-F:198 — Жесткий:383
441. Болт ГОСТ Р 50274-92 M8-6g×16-F:199 — Жесткий:384
442. Болт ГОСТ Р 50274-92 M8-6g×16-F:200 — Жесткий:385
443. Болт ГОСТ Р 50274-92 M8-6g×16-F:201 — Жесткий:386
444. Болт ГОСТ Р 50274-92 M8-6g×16-F:202 — Жесткий:387
445. Болт ГОСТ Р 50274-92 M8-6g×16-F:203 — Жесткий:388
446. Болт ГОСТ Р 50274-92 M8-6g×16-F:204 — Жесткий:389
447. Болт ГОСТ Р 50274-92 M8-6g×16-F:205 — Жесткий:390
448. Болт ГОСТ Р 50274-92 M8-6g×16-F:206 — Жесткий:391
449. Болт ГОСТ Р 50274-92 M8-6g×16-F:207 — Жесткий:392
450. Болт ГОСТ Р 50274-92 M8-6g×16-F:208 — Жесткий:393
451. Болт ГОСТ Р 50274-92 M8-6g×16-F:209 — Жесткий:394
452. Болт ГОСТ Р 50274-92 M8-6g×16-F:210 — Жесткий:395
453. Болт ГОСТ Р 50274-92 M8-6g×16-F:211 — Жесткий:396
454. Болт ГОСТ Р 50274-92 M8-6g×16-F:212 — Жесткий:397
455. Болт ГОСТ Р 50274-92 M8-6g×16-F:213 — Жесткий:398
456. Болт ГОСТ Р 50274-92 M8-6g×16-F:214 — Жесткий:399
457. Болт ГОСТ Р 50274-92 M8-6g×16-F:215 — Жесткий:400
458. Болт ГОСТ Р 50274-92 M8-6g×16-F:216 — Жесткий:401
459. Болт ГОСТ Р 50274-92 M8-6g×16-F:217 — Жесткий:402
460. Болт ГОСТ Р 50274-92 M8-6g×16-F:218 — Жесткий:403
461. Маслоотражательное кольцо_CPY:1 — Жесткий:404
462. Шпилька ГОСТ 22038-76 M20-6g×85:1 — Жесткий:126, Жесткий:125
463. Шайба ГОСТ 10450-78 21:1 — Жесткий:126
464. Гайка ГОСТ 15524-70 M20:1 — Жесткий:127
465. Шпилька ГОСТ 22038-76 M20-6g×85:4
466. Шайба ГОСТ 10450-78 21:2
467. Гайка ГОСТ 15524-70 M20:4
468. Шпилька ГОСТ 22038-76 M20-6g×85:5
469. Шайба ГОСТ 10450-78 21:3
470. Гайка ГОСТ 15524-70 M20:5
471. Шпилька ГОСТ 22038-76 M20-6g×85:6
472. Шайба ГОСТ 10450-78 21:4
473. Гайка ГОСТ 15524-70 M20:6
474. Шпилька ГОСТ 22038-76 M20-6g×85:7
475. Шайба ГОСТ 10450-78 21:5
476. Гайка ГОСТ 15524-70 M20:7
477. Шпилька ГОСТ 22038-76 M20-6g×85:8
478. Шайба ГОСТ 10450-78 21:6
479. Гайка ГОСТ 15524-70 M20:8
480. Шпилька ГОСТ 22038-76 M20-6g×85:9
481. Шайба ГОСТ 10450-78 21:7
482. Гайка ГОСТ 15524-70 M20:9
483. Шпилька ГОСТ 22038-76 M20-6g×85:10
484. Шайба ГОСТ 10450-78 21:8
485. Гайка ГОСТ 15524-70 M20:10
486. Шпилька ГОСТ 22038-76 M20-6g×85:11
487. Шайба ГОСТ 10450-78 21:9
488. Гайка ГОСТ 15524-70 M20:11
489. Шпилька ГОСТ 22038-76 M20-6g×85:12
490. Шайба ГОСТ 10450-78 21:10
491. Гайка ГОСТ 15524-70 M20:12
492. Шпилька ГОСТ 22038-76 M20-6g×85:13
493. Шайба ГОСТ 10450-78 21:11
494. Гайка ГОСТ 15524-70 M20:13
495. Шпилька ГОСТ 22038-76 M20-6g×85:14
496. Шайба ГОСТ 10450-78 21:12
497. Гайка ГОСТ 15524-70 M20:14
498. Шпилька ГОСТ 22038-76 M20-6g×85:15
499. Шайба ГОСТ 10450-78 21:13
500. Гайка ГОСТ 15524-70 M20:15
501. Шпилька ГОСТ 22038-76 M20-6g×85:16
502. Шайба ГОСТ 10450-78 21:14
503. Гайка ГОСТ 15524-70 M20:16
504. Шпилька ГОСТ 22038-76 M20-6g×85:17
505. Шайба ГОСТ 10450-78 21:15
506. Гайка ГОСТ 15524-70 M20:17
507. Шпилька ГОСТ 22038-76 M20-6g×85:18
508. Шайба ГОСТ 10450-78 21:16
509. Гайка ГОСТ 15524-70 M20:18
510. Гайка ГОСТ 15521-70 M20:1 — Жесткий:121
511. Шпилька ГОСТ 22034-76 M20-6g×50:1 — Жесткий:119, Жесткий:121, Жесткий:120
512. Шайба ГОСТ 10450-78 19:1 — Жесткий:120
513. Гайка ГОСТ 15521-70 M20:5
514. Шпилька ГОСТ 22034-76 M20-6g×50:5
515. Шайба ГОСТ 10450-78 19:5
516. Гайка ГОСТ 15521-70 M20:6
517. Шпилька ГОСТ 22034-76 M20-6g×50:6
518. Шайба ГОСТ 10450-78 19:6
519. Гайка ГОСТ 15521-70 M20:7
520. Шпилька ГОСТ 22034-76 M20-6g×50:7
521. Шайба ГОСТ 10450-78 19:7
522. Гайка ГОСТ 15521-70 M20:8
523. Шпилька ГОСТ 22034-76 M20-6g×50:8
524. Шайба ГОСТ 10450-78 19:8
525. Гайка ГОСТ 15521-70 M20:9
526. Шпилька ГОСТ 22034-76 M20-6g×50:9
527. Шайба ГОСТ 10450-78 19:9
528. Гайка ГОСТ 15521-70 M20:10
529. Шпилька ГОСТ 22034-76 M20-6g×50:10
530. Шайба ГОСТ 10450-78 19:10
531. Гайка ГОСТ 15521-70 M20:11
532. Шпилька ГОСТ 22034-76 M20-6g×50:11
533. Шайба ГОСТ 10450-78 19:11
534. Гайка ГОСТ 15521-70 M20:12
535. Шпилька ГОСТ 22034-76 M20-6g×50:12
536. Шайба ГОСТ 10450-78 19:12
537. Гайка ГОСТ 15521-70 M20:13
538. Шпилька ГОСТ 22034-76 M20-6g×50:13
539. Шайба ГОСТ 10450-78 19:13
540. Шпилька ГОСТ 22038-76 M24-6g×70:1 — Жесткий:113, Жесткий:111
541. Гайка ГОСТ 15524-70 M24:1 — Жесткий:113
542. Шайба  ГОСТ 11371-78 25:1 — Заподлицо:1, Жесткий:112
543. Шпилька ГОСТ 22038-76 M24-6g×70:18
544. Гайка ГОСТ 15524-70 M24:38
545. Шайба  ГОСТ 11371-78 25:18
546. Шпилька ГОСТ 22038-76 M24-6g×70:19
547. Гайка ГОСТ 15524-70 M24:39
548. Шайба  ГОСТ 11371-78 25:19
549. Шпилька ГОСТ 22038-76 M24-6g×70:20
550. Гайка ГОСТ 15524-70 M24:40
551. Шайба  ГОСТ 11371-78 25:20
552. Шпилька ГОСТ 22038-76 M24-6g×70:21
553. Гайка ГОСТ 15524-70 M24:41
554. Шайба  ГОСТ 11371-78 25:21
555. Шпилька ГОСТ 22038-76 M24-6g×70:22
556. Гайка ГОСТ 15524-70 M24:42
557. Шайба  ГОСТ 11371-78 25:22
558. Шпилька ГОСТ 22038-76 M24-6g×70:23
559. Гайка ГОСТ 15524-70 M24:43
560. Шайба  ГОСТ 11371-78 25:23
561. Шпилька ГОСТ 22038-76 M24-6g×70:24
562. Гайка ГОСТ 15524-70 M24:44
563. Шайба  ГОСТ 11371-78 25:24
564. Шпилька ГОСТ 22038-76 M24-6g×70:25
565. Гайка ГОСТ 15524-70 M24:45
566. Шайба  ГОСТ 11371-78 25:25
567. Шпилька ГОСТ 22038-76 M24-6g×70:26
568. Гайка ГОСТ 15524-70 M24:46
569. Шайба  ГОСТ 11371-78 25:26
570. Шпилька ГОСТ 22038-76 M24-6g×70:27
571. Гайка ГОСТ 15524-70 M24:47
572. Шайба  ГОСТ 11371-78 25:27
573. Шпилька ГОСТ 22038-76 M24-6g×70:28
574. Гайка ГОСТ 15524-70 M24:48
575. Шайба  ГОСТ 11371-78 25:28
576. Шпилька ГОСТ 22038-76 M24-6g×70:29
577. Гайка ГОСТ 15524-70 M24:49
578. Шайба  ГОСТ 11371-78 25:29
579. Шпилька ГОСТ 22038-76 M24-6g×70:30
580. Гайка ГОСТ 15524-70 M24:50
581. Шайба  ГОСТ 11371-78 25:30
582. Шпилька ГОСТ 22038-76 M24-6g×70:31
583. Гайка ГОСТ 15524-70 M24:51
584. Шайба  ГОСТ 11371-78 25:31
585. Шпилька ГОСТ 22038-76 M24-6g×70:32
586. Гайка ГОСТ 15524-70 M24:52
587. Шайба  ГОСТ 11371-78 25:32
588. Винт ГОСТ 11738-84 M 10x35:1 — Жесткий:129
589. Шайба  ГОСТ 11371-78 13:1 — Жесткий:128, Жесткий:129
590. Винт ГОСТ 11738-84 M 10x35:2
591. Шайба  ГОСТ 11371-78 13:5